# Autodesk Inventor assembly: 043.5-HRPK
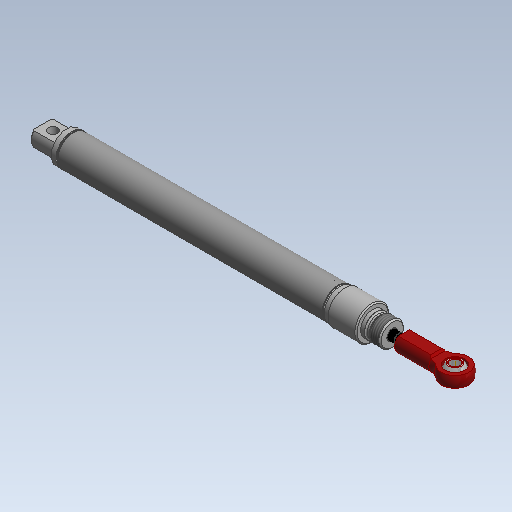
[picture p0: Inventor's stored thumbnail of the model, 512x512]
Saved by Autodesk Inventor 2020 (Build 240168000, 168)
## iProperties
Part Number: 043.5-HRPK
Catalog Web Link: www.cadenas.de
Description: Original Line Standard Air Cylinders-Standard Air Cylinders
Vendor: BIMBA
Document SubType Name: Assembly
Designer: partserver
Manufacturer: BIMBA
Mass: 56.7382 g
Surface Area: 392.845 cm^2
Volume: 50.4942 cm^3
Density: 1.12366 g/cm^3
Category: PARTsolutions
Company: BIMBA
PSOL_IDENT_0: {$CADENAS_DATA\23d-libs\bimba\bimba_brand\bimba_imperial\bimba_full_line\original_line_cylinders\sta
PSOL_IDENT_1: ndard_air_cylinders\standard_air_cylinder_asmtab.prj},328 {VTYP=3D},{STYP=ASSTAB},{NB=043.5-HRPK},{L
PSOL_IDENT_2: INA=043.5-HRPK},{NN=Original Line Standard Air Cylinders},{DATE=19.01.2022 10:19:38},{GEOMDATE=11.11
PSOL_IDENT_3: .2021 07:31:43},{VERSION=},{LINEID=50},{WBVAR=STROKE,ACTING,MNT,DER,NR,BM,CO,OO,VO,M,EE,EEL,K,Q,Y,G,
PSOL_IDENT_4: T,HL,B,H,SER,SR,NT,W,STPT1,STPT2,STPT3,STPT4,MB,PB,PRC,TB,MN},{WBNUMERIC=STROKE,EEL}  {NB=043.5-HRPK
PSOL_IDENT_5: },{LINA=043.5-HRPK},{KT=DUMMY},{PN=043.5-HRPK},{PNC=043.5-HRPK},{PNA=(NO ACCESSORIES)},{PNAHELP=},{D
PSOL_IDENT_6: ASH=-},{BORE1=0.75000000},{BORE=3/4\" (04)},{BOREPN=04},{STROKE=3.500},{STROKEALG=[0.011:50/0.001]},
PSOL_IDENT_7: {STROKE1=3.500},{ACTING=R},{ACTINGALG= '' , 'Single Acting' , 'R' , 'Reverse Single Acting (R)' , 'D'
PSOL_IDENT_8: , 'Double Acting (D)' },{ACTINGPN=R},{MNT=P},{MNTALG= '' , 'Front Nose Mounting' , 'P' , 'Rear Pivo
PSOL_IDENT_9: t Mounting (P)' , 'BF' , 'Front Block Mounting (BF)' , 'BR' , 'Rear Block Mounting for Vertical Posi
PSOL_IDENT_10: tioning (BR)' , 'A' , 'Nose Mounting with Adjustable Stroke (A)' },{TYPE=},{MNTPN=P},{DER=},{DERALG=
PSOL_IDENT_11: '' , 'N/A' },{NR=},{NRALG= '' , 'N/A' },{NRPN=},{BM=},{BMALG= '' , 'N/A' },{BMPN=},{CO=},{COALG= ''
PSOL_IDENT_12: , 'N/A' },{OO=},{OOALG= '', 'N/A' },{OOPN=},{VO=Z},{VOALG= 'Z' , 'N/A' },{VOPN=},{OOVOPN=},{M=},{MA
PSOL_IDENT_13: LG= '', 'Without Magnet', 'M', 'With Magnet' },{EE=},{EEL=0.000},{EEMAX=46.5000},{EEALG= '', 'Withou
PSOL_IDENT_14: t Extra Extension', 'EE', 'With Extra Extension' },{EELALG=0},{EEPN=},{EEPN1=0.000},{K=K},{KALG= '',
PSOL_IDENT_15: 'Standard' , 'K' , 'Ports Rotated 90deg K' },{KPN=K},{Q=},{QALG= '' , 'N/A' },{QPN=},{Y=},{YALG= ''
PSOL_IDENT_16: , 'Without Pivot Bushing' , 'Y' , 'With Pivot Bushing' },{YPN=},{YCON=},{F=},{FALG= '', 'Non-Coated
PSOL_IDENT_17: (Standard)', 'F', 'Molycoated' },{FPN=},{G=},{GPN=},{GPN99=},{T=},{TALG= '' , 'Standard -20° to 200
PSOL_IDENT_18: °F (-29° to 95°C)' , 'N' , 'Low Temperature' , 'V' , 'High Temperature' },{NPN=},{VPN=},{HL=},{HLALG=
PSOL_IDENT_19: '' , 'N/A' },{B=},{BALG= '', 'W/out Bumpers' , 'B' , 'W/ Bumpers' },{BPN=},{H=H},{HALG= '', 'W/ Sta
PSOL_IDENT_20: ndard Spring (Relaxed 3 lbs./Compressed 6 lbs.)', 'H', 'W/ Heavy Spring (Relaxed 4 lbs./Compressed 1
PSOL_IDENT_21: 0 lbs.)' },{HPN=H},{SER=},{SERALG= '' , 'N/A' },{SR=C},{SRALG= 'C' , 'Standard Blackened Carbon Stee
PSOL_IDENT_22: l' , 'SR' , 'Stainless Steel [SR]' },{SRPN=},{SRCON=1},{NT=},{NTPN=},{W=},{WALG= '' , 'N/A' },{WPN=}
PSOL_IDENT_23: ,{E=},{EALG= '' , 'Standard Seals/Lube' , 'E' , 'Non-Lube Seals/Lube' },{EPN=},{ST=},{STALG= '' , 'N
PSOL_IDENT_24: /A' },{STPT1=},{STPT1ALG= '' , 'N/A' },{STPT2=},{STPT2ALG= '' , 'N/A' },{STPT3=},{STPT3ALG= '' , 'N/
PSOL_IDENT_25: A' },{STPT4=},{STPT4ALG= '' , 'N/A' },{STPN=},{MB=},{MBALG= '' , 'N/A' },{MBPN=},{MBPNALL=},{MBPNALL
PSOL_IDENT_26: REAR=},{PB=},{PBALG= '' , 'Without Pivot Bracket' , 'D-167' , 'D-167' },{PBPN=},{PBPNALL=D-167},{PRC=
PSOL_IDENT_27: },{PRCALG= '' , 'W/out Pivot Rod Clevis' , 'F,D-166-3' , 'D-166-3 (front)' },{PRCPN=},{PRCPNALL=D-16
PSOL_IDENT_28: 6-3},{TB=},{TBALG= '' , 'N/A' },{TBPN=},{TBPNALL=},{MN=},{MNALG= '' , 'Without Mounting Nut' , 'F,D-
PSOL_IDENT_29: 9' , 'D-9 (front)' },{MNPN=},{MNCONF=},{MNCONR=},{TLEN=6.8295},{FRAC=12.2000},{RGCON=},{RGDACCON=R},
PSOL_IDENT_30: {RHCON=P},{RHCON1=P},{RHCONON=1},{RHACCON=R},{FNUTCON=0},{RNUTCON=0},{FNUTPN=D-9},{RNUTPN=},{FNUTTRA
PSOL_IDENT_31: NS=0.0000},{RNUTTRANS=0.0000},{VHOLECON=3},{A1=1.5940},{A1N=0.8750},{A1P=1.5940},{A1B=1.5940},{A4=0.
PSOL_IDENT_32: 2525},{A4N=0.3130},{A4P=0.2525},{A5=0.0300},{A1H=0.2785},{A1NH=0.5310},{A1PH=1.5940},{A1BH=1.0940},{
PSOL_IDENT_33: A1SH=1.2190},{A2H=0.1560},{A2NH=0.2190},{LENGTH=2.4400},{LENGTH1=2.4400},{LENGTH2=3.8100},{MUL=9.415
PSOL_IDENT_34: 0},{MUL11=9.4150},{MUL22=9.415},{MUL33=5.9150},{MUL2=2.6900},{MUL211=2.6900},{MUL222=2.6900},{MUL233=
PSOL_IDENT_35: 1.6900},{SSS=7.0000},{RGLEN=1.3715},{RHLEN=0.4990},{SSS1=4.0000},{A13=1.3120},{DIF=0.0000},{G5=0.625
PSOL_IDENT_36: 0},{ON=1},{SSADD=0.0000},{BADD=0.0000},{MADD=0.0000},{NVADD=0.0000},{TRACKL=6.5395},{TRACKCON=D-7416
PSOL_IDENT_37: 8},{TRIMCON=0},{TRIMCON1=0},{PINCON=D-51},{FSPACE=0.5770},{SPACE=0.0804},{TEXT=0.1406},{S1=1.0000},{
PSOL_IDENT_38: D1=0.8325},{D1N=0.8050},{D1B=0.8625},{D1P=0.8325},{FA=0.940},{RA=0.9400},{PPATH=standard_air_cylinde
PSOL_IDENT_39: r_asmtpl.prj},{MATALGHTML=<b>Standard Original Line:</b><dl><dt>Rod:</dt><dd>- Stainless Steel</dd><
PSOL_IDENT_40: dd>&nbsp;&nbsp;(5/16 9/16 Bores)</dd><dd>- High Strength Carbon Steel</dd><dd>&nbsp;&nbsp;(3/4 3 Bor
PSOL_IDENT_41: e)</dd><dd>- Stainless Steel</dd><dd>&nbsp;&nbsp;(X style DXP/DX/DXDE)</dd><dt>Bearings:</dt><dd>- S
PSOL_IDENT_42: intered Bronze</dd><dt>Body:</dt><dd>- 304 Stainless Steel</dd><dt>End Caps:</dt><dd>- Aluminum</dd>
PSOL_IDENT_43: <dt>Seals:</dt><dd>- Buna N</dd></dl>},{ASSCFGPRA=04RP},{MBPNA=},{MNPNA=},{PRCPNA=},{ASSOPTACC=STPT4
PSOL_IDENT_44: },{A=12.20},{HADD=0.0000},{WFL=0.25},{QADD=0.000},{QADD1=0.440},{TEST=3.0000},{MNTB=},{STDNUTF=0},{S
PSOL_IDENT_45: TDNUTR=0},{STRK2D=0},{X2D=2},{STROKESW=3.500},{EESW=0.000},{FCD=0},{BCD=0},{RCD=0},{CUSTADD=2.500},{
PSOL_IDENT_46: FT=1/4-28 UNF-2A},{FT1=1/4-28 UNF-2A},{FT2=1/2-20 UNF-2A},{PORT=1/8 NPT},{FT11=1/2-20 UNF-2A},{FT12=
PSOL_IDENT_47: 5/8-18 UNF-2A},{B1=}
NB: 043.5-HRPK
NN: Original Line Standard Air Cylinders
NT: Threaded (Standard)
NBSYN: $PNC.
LINA: 043.5-HRPK
CATALOG: Bimba Products
PN: 043.5-HRPK
PNA: (NO ACCESSORIES)
BORE: 3/4" (04)
STROKE: 3.5
ACTING: Reverse Single Acting (R)
MNT: Rear Pivot Mounting (P)
DER: N/A
NR: N/A
BM: N/A
CO: N/A
OO: N/A
VO: N/A
M: Without Magnet
EE: Without Extra Extension
EEL: 0
K: Ports Rotated 90deg K
Q: N/A
Y: Without Pivot Bushing
G: Standard Lube
T: Standard -20° to 200°F (-29° to 95°C)
HL: N/A
B: W/out Bumpers
H: W/ Heavy Spring (Relaxed 4 lbs./Compressed 10 lbs.)
SER: N/A
SR: Standard Blackened Carbon Steel
W: N/A
STPT1: N/A
STPT2: N/A
STPT3: N/A
STPT4: N/A
MB: N/A
PB: Without Pivot Bracket
PRC: W/out Pivot Rod Clevis
TB: N/A
MN: Without Mounting Nut
A: 12.2
SUPPLIER: BIMBA
ARTICLENO: 043.5-HRPK
BOMINFO: 043.5-HRPK
CREATOR: CADENAS GmbH
Title: 043.5-HRPK
Author: Cadenas PARTsolutions
Comments: Standard Air Cylinders
## Documents named in this file (7)
- T:\EIT\2022 Rapid React\COMMON PARTS\AIR CYLINDERS\BIMBA_0435HRPK\AIS2020\043_5-HRPK.iam
- T:\EIT\2022 Rapid React\COMMON PARTS\AIR CYLINDERS\BIMBA_0435HRPK\AIS2020\043_5-HRPCK0000000_0_dummy.ipt
- T:\EIT\2022 Rapid React\COMMON PARTS\AIR CYLINDERS\BIMBA_0435HRPK\AIS2020\04RK000-3_5_rod_guide.ipt
- T:\EIT\2022 Rapid React\COMMON PARTS\AIR CYLINDERS\BIMBA_0435HRPK\AIS2020\04R-6_82953C.ipt
- T:\EIT\2022 Rapid React\COMMON PARTS\AIR CYLINDERS\BIMBA_0435HRPK\AIS2020\04PR0K000_rear_head.ipt
- T:\EIT\2022 Rapid React\COMMON PARTS\AIR CYLINDERS\BIMBA_0435HRPK\AIS2020\C-043_5-HRP0000_rod.ipt
- T:\EIT\2022 Rapid React\COMMON PARTS\AIR CYLINDERS\TieRod End\60685K321_PTFE-LINED ALUMINUM BALL JOINT ROD END.ipt
## Components (6 placed, 6 different names)
1. 043_5-HRPCK0000000_0_dummy:1
2. 04RK000-3_5_rod_guide:1 — Insert:1
3. 04R-6_82953C:1
4. 04PR0K000_rear_head:1 — Angle:1
5. C-043_5-HRP0000_rod:1 — Insert:1, Insert:2
6. 60685K321_PTFE-LINED ALUMINUM BALL JOINT ROD END:1 — Insert:2, Angle:1
## Relationships (3: Insert 2, Angle 1)
- Insert:1: 04RK000-3_5_rod_guide:1 ↔ C-043_5-HRP0000_rod:1
- Insert:2 (-3 mm): C-043_5-HRP0000_rod:1 ↔ 60685K321_PTFE-LINED ALUMINUM BALL JOINT ROD END:1
- Angle:1 (0 deg): 04PR0K000_rear_head:1 ↔ 60685K321_PTFE-LINED ALUMINUM BALL JOINT ROD END:1
